# Autodesk Inventor assembly: czlon_1
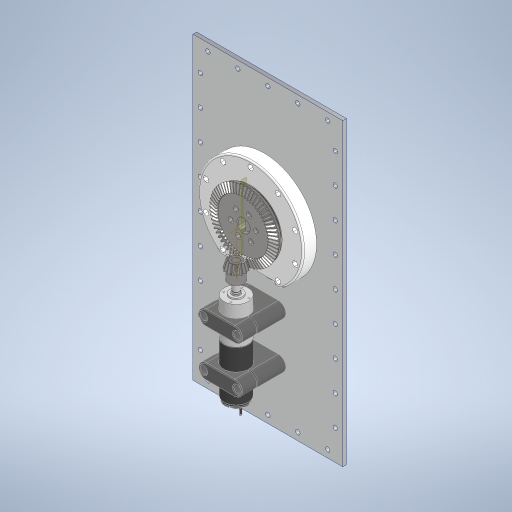
[picture p0: Inventor's stored thumbnail of the model, 512x512]
Saved by Autodesk Inventor 2023 (Build 270158000, 158)
## iProperties
Created: 2023-04-11
Part Number: czlon_1
Document SubType Name: Assembly
Designer: Kamil
Author: Kamil
## Documents named in this file (8)
- C:\Users\Kamil\Desktop\KONARM_2\czlon 2\czlon_1.iam
- C:\Users\Kamil\Desktop\KONARM_2\czlon 1\32010-X-GY-002.ipt
- C:\Users\Kamil\Desktop\KONARM_2\czlon 1\Faulhaber 3272G012C R.ipt
- C:\Users\Kamil\Desktop\KONARM_2\czlon 1\podst.ipt
- C:\Users\Kamil\Desktop\KONARM_2\czlon 1\Podstawa.ipt
- C:\Users\Kamil\Desktop\KONARM_2\czlon 1\Uchwyt_silnika_2_dół.ipt
- C:\Users\Kamil\Desktop\KONARM_2\czlon 1\Uchwyt_silnika_2_góra.ipt
- C:\Users\Kamil\Desktop\KONARM_2\czlon 1\Assembly3\Design Accelerator\Bevel Gears1.iam
## Components (10 placed, 7 different names)
1. 32010-X-GY-002:1 — Zestawiające:4, Zestawiające:5, Zestawiające:7
2. Faulhaber 3272G012C R:1 — Zestawiające:14, Zestawiające:15, Zestawiające:18, Zestawiające:21
3. podst:1 — Zestawiające:1, Zestawiające:2, Zestawiające:3, Zestawiające:22
4. Podstawa:1 — Zestawiające:1, Zestawiające:2, Zestawiające:3, Zestawiające:4, Zestawiające:5, Zestawiające:6, Zestawiające:8, Zestawiające:9, Zestawiające:10, Zestawiające:11, Zestawiające:12, Zestawiające:13, Zestawiające:20
5. Uchwyt_silnika_2_dół:1 — Zestawiające:18, Zestawiające:19, Zestawiające:20
6. Uchwyt_silnika_2_góra:1 — Zestawiające:9, Zestawiające:11, Zestawiające:13, Zestawiające:14, Zestawiające:19
7. Uchwyt_silnika_2_dół:2 — Zestawiające:15, Zestawiające:16, Zestawiające:17
8. Uchwyt_silnika_2_góra:2 — Zestawiające:8, Zestawiające:10, Zestawiające:12, Zestawiające:16, Zestawiające:17
9. 32010-X-GY-002:2 — Zestawiające:6, Zestawiające:7
10. Bevel Gears:1 [sub-assembly] — Zestawiające:21, Zestawiające:22
## Relationships (22: Mate 22)
- Zestawiające:1 [Mate]: podst:1 ↔ Podstawa:1
- Zestawiające:2 [Mate]: podst:1 ↔ Podstawa:1
- Zestawiające:3 [Mate]: podst:1 ↔ Podstawa:1
- Zestawiające:4 [Mate]: 32010-X-GY-002:1 ↔ Podstawa:1
- Zestawiające:5 [Mate]: 32010-X-GY-002:1 ↔ Podstawa:1
- Zestawiające:6 [Mate]: Podstawa:1 ↔ 32010-X-GY-002:2
- Zestawiające:7 [Mate]: 32010-X-GY-002:1 ↔ 32010-X-GY-002:2
- Zestawiające:8 [Mate]: Podstawa:1 ↔ Uchwyt_silnika_2_góra:2
- Zestawiające:9 [Mate]: Podstawa:1 ↔ Uchwyt_silnika_2_góra:1
- Zestawiające:10 [Mate]: Podstawa:1 ↔ Uchwyt_silnika_2_góra:2
- Zestawiające:11 [Mate]: Podstawa:1 ↔ Uchwyt_silnika_2_góra:1
- Zestawiające:12 [Mate]: Podstawa:1 ↔ Uchwyt_silnika_2_góra:2
- Zestawiające:13 [Mate]: Podstawa:1 ↔ Uchwyt_silnika_2_góra:1
- Zestawiające:14 [Mate]: Faulhaber 3272G012C R:1 ↔ Uchwyt_silnika_2_góra:1
- Zestawiające:15 [Mate]: Faulhaber 3272G012C R:1 ↔ Uchwyt_silnika_2_dół:2
- Zestawiające:16 [Mate]: Uchwyt_silnika_2_dół:2 ↔ Uchwyt_silnika_2_góra:2
- Zestawiające:17 [Mate]: Uchwyt_silnika_2_dół:2 ↔ Uchwyt_silnika_2_góra:2
- Zestawiające:18 [Mate]: Faulhaber 3272G012C R:1 ↔ Uchwyt_silnika_2_dół:1
- Zestawiające:19 [Mate]: Uchwyt_silnika_2_dół:1 ↔ Uchwyt_silnika_2_góra:1
- Zestawiające:20 [Mate]: Podstawa:1 ↔ Uchwyt_silnika_2_dół:1
- Zestawiające:21 [Mate]: Faulhaber 3272G012C R:1 ↔ Bevel Gears:1
- Zestawiające:22 [Mate]: podst:1 ↔ Bevel Gears:1
